# Autodesk Inventor assembly: MicromouseAssembly
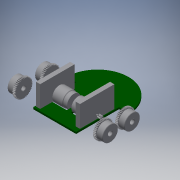
[picture p0: Inventor's stored thumbnail of the model, 180x180]
Saved by Autodesk Inventor 2018 (Build 220112000, 112)
## iProperties
Created: 2017-09-20
Part Number: MicromouseAssembly
Document SubType Name: Assembly
Designer: Yikealo
Author: Yikealo
## Documents named in this file (6)
- D:\micromous model\MicromouseAssembly.iam
- D:\micromous model\Micromouse_pcb.ipt
- D:\micromous model\motor.ipt
- D:\micromous model\spur_gear_motor.ipt
- D:\micromous model\spur_gear_wheels_40T.ipt
- D:\micromous model\mounting.ipt
## Components (11 placed, 5 different names)
1. Micromouse1.2.kicad_pcb:1 — Mate:1, Mate:2, Mate:5, Mate:6
2. motor:1 — Mate:2, Mate:3, Flush:1, Flush:3, Mate:7, Mate:8
3. motor:2 — Mate:1, Mate:4, Flush:2, Flush:4, Mate:7, Mate:8
4. spur_gear_motor:1 — Mate:3, Flush:1
5. spur_gear_motor:2 — Mate:4, Flush:2
6. spur_gear_wheels_40T:1
7. spur_gear_wheels_40T:2
8. spur_gear_wheels_40T:3
9. spur_gear_wheels_40T:4
10. mounting:1 — Mate:5, Flush:4
11. mounting:2 — Mate:6, Flush:3
## Relationships (12: Mate 8, Flush 4)
- Mate:1: Micromouse1.2.kicad_pcb:1 ↔ motor:2
- Mate:2: Micromouse1.2.kicad_pcb:1 ↔ motor:1
- Mate:3: motor:1 ↔ spur_gear_motor:1
- Flush:1: motor:1 ↔ spur_gear_motor:1
- Mate:4: motor:2 ↔ spur_gear_motor:2
- Flush:2: motor:2 ↔ spur_gear_motor:2
- Mate:5: Micromouse1.2.kicad_pcb:1 ↔ mounting:1
- Mate:6: Micromouse1.2.kicad_pcb:1 ↔ mounting:2
- Flush:3: motor:1 ↔ mounting:2
- Flush:4: motor:2 ↔ mounting:1
- Mate:7: motor:1 ↔ motor:2
- Mate:8: motor:1 ↔ motor:2
